# Autodesk Inventor assembly: Property
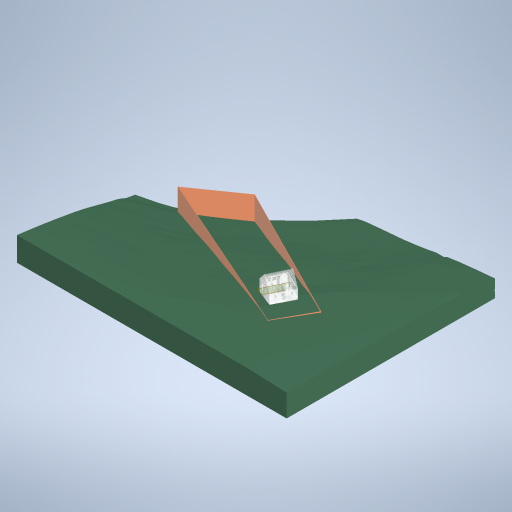
[picture p0: Inventor's stored thumbnail of the model, 512x512]
Saved by Autodesk Inventor 2024 (Build 280153020, 153B)
## iProperties
Created: 2023-06-05
Part Number: Property
Document SubType Name: Assembly
Designer: Tom
Author: Tom
## Documents named in this file (4)
- C:\Users\Tom\Documents\Tom_Levers_Public_Git_Repository\Inventor\Mobility\Property.iam
- C:\Users\Tom\Documents\Tom_Levers_Public_Git_Repository\Inventor\Mobility\Land.ipt
- C:\Users\Tom\Documents\Tom_Levers_Public_Git_Repository\Inventor\Mobility\Fence.ipt
- C:\Users\Tom\Documents\Tom_Levers_Public_Git_Repository\Inventor\Mobility\Finished_House.iam
## Components (3 placed, 3 different names)
1. Land:1 — Flush:1, Mate:1, Mate:2
2. Fence:1
3. Finished_House:1 [sub-assembly] — Flush:1, Mate:1, Mate:2
## Relationships (3: Mate 2, Flush 1)
- Flush:1 (6248.4 mm): Land:1 ↔ Finished_House:1
- Mate:1 (12.7 mm): Land:1 ↔ Finished_House:1
- Mate:2 (228.6 mm): Land:1 ↔ Finished_House:1
